# Autodesk Inventor assembly: assyEscapement
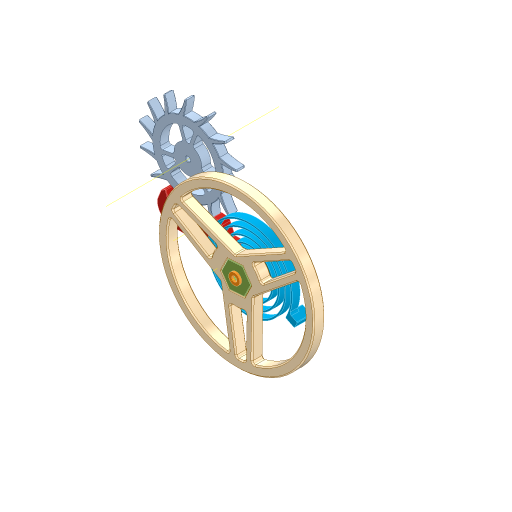
[picture p0: Inventor's stored thumbnail of the model, 512x512]
Saved by Autodesk Inventor 2023 (Build 270158000, 158)
## iProperties
Created: 2023-02-14
Part Number: assyEscapement
Document SubType Name: Assembly
Designer: Aditya
Author: Aditya
## Documents named in this file (4)
- C:\Users\Aditya\Documents\Inventor\Tourbillon\assyEscapement.iam
- C:\Users\Aditya\Documents\Inventor\Tourbillon\escapement.ipt
- C:\Users\Aditya\Documents\Inventor\Tourbillon\balanceWheel.ipt
- C:\Users\Aditya\Documents\Inventor\Tourbillon\washer.ipt
## Components (9 placed, 3 different names)
1. escapement:1 — Flush:1, Flush:2, Flush:3, Mate:1, Flush:4, Mate:2, Rigid:1, Rigid:2, Rigid:6
2. balanceWheel:1 — Mate:1, Flush:4, Angle:1, Mate:2, Rigid:3, Rigid:4
3. washer:1 — Rigid:1
4. washer:2 — Rigid:2
5. washer:3 — Rotational:1
6. washer:4 — Rotational:1, Rigid:3
7. washer:5 — Rigid:4, Rigid:5
8. washer:6 — Rigid:5
9. washer:7 — Rigid:6
## Relationships (14: WeldJoint 6, Flush 4, Mate 2, Angle 1, RevoluteJoint 1)
- Flush:1: escapement:1
- Flush:2: escapement:1
- Flush:3: escapement:1
- Mate:1: escapement:1 ↔ balanceWheel:1
- Flush:4: escapement:1 ↔ balanceWheel:1
- Angle:1 (28 deg): balanceWheel:1
- Mate:2: escapement:1 ↔ balanceWheel:1
- Rigid:1 [WeldJoint]: escapement:1 ↔ washer:1
- Rigid:2 [WeldJoint]: escapement:1 ↔ washer:2
- Rotational:1 [RevoluteJoint]: washer:3 ↔ washer:4
- Rigid:3 [WeldJoint]: balanceWheel:1 ↔ washer:4
- Rigid:4 [WeldJoint]: balanceWheel:1 ↔ washer:5
- Rigid:5 [WeldJoint]: washer:5 ↔ washer:6
- Rigid:6 [WeldJoint]: escapement:1 ↔ washer:7
